# Autodesk Inventor assembly: 2f2
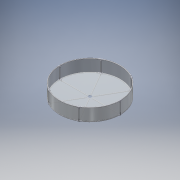
[picture p0: Inventor's stored thumbnail of the model, 180x180]
Saved by Autodesk Inventor 2016 (Build 200138000, 138)
## iProperties
Company: HERA Project
Created: 2013-06-27
Part Number: 2f2
Document SubType Name: Assembly
Designer: David DeBoer
Description: Feed backplane support assembly
Author: David DeBoer
Title: Feed backplane support
## Documents named in this file (9)
- C:\Users\ddeboer\Desktop\hera-cad\feed\bpScreenAssembly.iam
- C:\Users\ddeboer\Desktop\hera-cad\feed\bpSupArm.ipt
- C:\Users\ddeboer\Desktop\hera-cad\smallParts\pvc_T_0.75in.ipt
- C:\Users\ddeboer\Desktop\hera-cad\feed\bpSupArc.ipt
- C:\Users\ddeboer\Desktop\hera-cad\jigs\bpSparJig.ipt
- C:\Users\ddeboer\Desktop\hera-cad\feed\bpSupVertArm.ipt
- C:\Users\ddeboer\Desktop\hera-cad\smallParts\angleBracketB.ipt
- C:\Users\ddeboer\Desktop\hera-cad\feed\bpScreen.ipt
- C:\Users\ddeboer\Desktop\hera-cad\feed\bpCylinder.ipt
## Components (45 placed, 8 different names)
1. bpSparJig:1 — Mate:1, Mate:2, Mate:3, Angle:3, Angle:4, Mate:9, Mate:11
2. bpScreen:1 — Mate:9, Angle:5, Mate:10, Tangent:1
3. bpCylinder:1 — Mate:10, Mate:11
4. bpSupArc:1 — Angle:4, Mate:13, Mate:14
5. pvc_T_0.75in:1 — Insert:1, Angle:1, Mate:4, Angle:2, Mate:12, Mate:13, Mate:14
6. bpSupArm:1 — Mate:1, Mate:2, Mate:3, Insert:1, Angle:1, Angle:6, Tangent:1
7. bpSupArc:7 — Angle:3, Mate:15, Mate:16
8. pvc_T_0.75in:7 — Insert:2, Angle:2, Mate:15, Mate:16
9. bpSupVertArm:1 — Mate:6, Mate:7, Mate:8, Insert:2
10. angleBracketB:1 — Mate:4, Mate:6, Mate:7, Mate:8, Angle:6, Mate:12
11. bpSupArc:8
12. pvc_T_0.75in:8
13. bpSupArm:2
14. bpSupArc:9
15. pvc_T_0.75in:9
16. bpSupVertArm:2
17. angleBracketB:2
18. bpSupArc:10
19. pvc_T_0.75in:10
20. bpSupArm:3
21. bpSupArc:11
22. pvc_T_0.75in:11
23. bpSupVertArm:3
24. angleBracketB:3
25. bpSupArc:12
26. pvc_T_0.75in:12
27. bpSupArm:4
28. bpSupArc:13
29. pvc_T_0.75in:13
30. bpSupVertArm:4
31. angleBracketB:4
32. bpSupArc:14
33. pvc_T_0.75in:14
34. bpSupArm:5
35. bpSupArc:15
36. pvc_T_0.75in:15
37. bpSupVertArm:5
38. angleBracketB:5 — Angle:5
39. bpSupArc:16
40. pvc_T_0.75in:16
41. bpSupArm:6
42. bpSupArc:17
43. pvc_T_0.75in:17
44. bpSupVertArm:6
45. angleBracketB:6
## Component patterns: (6 elements, first: bpSupArc:1 + pvc_T_0.75in:1 + bpSupArm:1 + bpSupArc:7 + pvc_T_0.75in:7 + bpSupVertArm:1 + angleBracketB:1)
## Relationships (24: Mate 15, Angle 6, Insert 2, Tangent 1)
- Mate:1: bpSparJig:1 ↔ bpSupArm:1
- Mate:2: bpSparJig:1 ↔ bpSupArm:1
- Mate:3: bpSparJig:1 ↔ bpSupArm:1
- Insert:1 (-39.5 mm): pvc_T_0.75in:1 ↔ bpSupArm:1
- Angle:1 (0 deg): pvc_T_0.75in:1 ↔ bpSupArm:1
- Mate:4: pvc_T_0.75in:1 ↔ angleBracketB:1
- Mate:6: bpSupVertArm:1 ↔ angleBracketB:1
- Mate:7: bpSupVertArm:1 ↔ angleBracketB:1
- Mate:8: bpSupVertArm:1 ↔ angleBracketB:1
- Insert:2 (-39.5 mm): pvc_T_0.75in:7 ↔ bpSupVertArm:1
- Angle:2 (0 deg): pvc_T_0.75in:1 ↔ pvc_T_0.75in:7
- Angle:3 (0 deg): bpSparJig:1 ↔ bpSupArc:7
- Angle:4 (0 deg): bpSparJig:1 ↔ bpSupArc:1
- Mate:9: bpSparJig:1 ↔ bpScreen:1
- Angle:5 (0 deg): bpScreen:1 ↔ angleBracketB:5
- Mate:10: bpScreen:1 ↔ bpCylinder:1
- Mate:11: bpSparJig:1 ↔ bpCylinder:1
- Angle:6 (0 deg): bpSupArm:1 ↔ angleBracketB:1
- Mate:12: pvc_T_0.75in:1 ↔ angleBracketB:1
- Mate:13: bpSupArc:1 ↔ pvc_T_0.75in:1
- Mate:14: bpSupArc:1 ↔ pvc_T_0.75in:1
- Mate:15: bpSupArc:7 ↔ pvc_T_0.75in:7
- Mate:16: bpSupArc:7 ↔ pvc_T_0.75in:7
- Tangent:1: bpScreen:1 ↔ bpSupArm:1
